# Autodesk Inventor assembly: EnsambleCuerpo
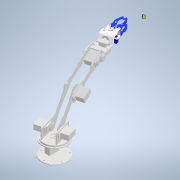
[picture p0: Inventor's stored thumbnail of the model, 180x180]
Saved by Autodesk Inventor 2022 (Build 260153000, 153)
## iProperties
Created: 2021-09-09
Part Number: EnsambleCuerpo
Document SubType Name: Assembly
Designer: Administrador
Author: Administrador
## Documents named in this file (19)
- C:\Users\Administrador\Desktop\Octavo Semestre\Robótica Industrial\Robot\Cuerpo\EnsambleCuerpo.iam
- C:\Users\Administrador\Desktop\Octavo Semestre\Robótica Industrial\Robot\Cuerpo\PartesCuerpo\Base_Suelo.ipt
- C:\Users\Administrador\Desktop\Octavo Semestre\Robótica Industrial\Robot\Cuerpo\PartesCuerpo\Base2.ipt
- C:\Users\Administrador\Desktop\Octavo Semestre\Robótica Industrial\Robot\Cuerpo\PartesCuerpo\Motor Mg995.ipt
- C:\Users\Administrador\Desktop\Octavo Semestre\Robótica Industrial\Robot\Cuerpo\PartesCuerpo\Base3.ipt
- C:\Users\Administrador\Desktop\Octavo Semestre\Robótica Industrial\Robot\Cuerpo\PartesCuerpo\Circulo_Inferior.ipt
- C:\Users\Administrador\Desktop\Octavo Semestre\Robótica Industrial\Robot\Cuerpo\PartesCuerpo\Base4.ipt
- C:\Users\Administrador\Desktop\Octavo Semestre\Robótica Industrial\Robot\Cuerpo\PartesCuerpo\BaseMotoresHombrp.ipt
- C:\Users\Administrador\Desktop\Octavo Semestre\Robótica Industrial\Robot\Cuerpo\PartesCuerpo\Brazo1.1.ipt
- C:\Users\Administrador\Desktop\Octavo Semestre\Robótica Industrial\Robot\Cuerpo\PartesCuerpo\Estella Servo1.ipt
- C:\Users\Administrador\Desktop\Octavo Semestre\Robótica Industrial\Robot\Cuerpo\PartesCuerpo\Brazo2Izquierda.ipt
- C:\Users\Administrador\Desktop\Octavo Semestre\Robótica Industrial\Robot\Cuerpo\PartesCuerpo\Brazo1Izquierda.ipt
- C:\Users\Administrador\Desktop\Octavo Semestre\Robótica Industrial\Robot\Cuerpo\PartesCuerpo\Brazo2Derecha.ipt
- C:\Users\Administrador\Desktop\Octavo Semestre\Robótica Industrial\Robot\Cuerpo\PartesCuerpo\Brazo3Izquierda.ipt
- C:\Users\Administrador\Desktop\Octavo Semestre\Robótica Industrial\Robot\Cuerpo\PartesCuerpo\Brazo3.ipt
- C:\Users\Administrador\Desktop\Octavo Semestre\Robótica Industrial\Robot\Cuerpo\PartesCuerpo\Muñeca1.ipt
- C:\Users\Administrador\Desktop\Octavo Semestre\Robótica Industrial\Robot\Cuerpo\PartesCuerpo\Muñeca2.ipt
- C:\Users\Administrador\Desktop\Octavo Semestre\Robótica Industrial\Robot\Cuerpo\PartesCuerpo\Microservo Mg90.ipt
- C:\Users\Administrador\Desktop\Octavo Semestre\Robótica Industrial\Robot\Pinza\Ensamble Pinza.iam
## Components (26 placed, 18 different names)
1. Base3:1 — Mate:6, Mate:7, Mate:8, Mate:9, Rigid:16, Mate:11, Mate:12
2. Circulo_Inferior:1 — Mate:7, Mate:8, Mate:9, Rigid:16, Rotational:1, Mate:10
3. Base4:1 — Mate:10, Mate:11, Mate:12, Mate:13, Mate:14, Mate:15
4. Base_Suelo:1 — Rigid:15
5. Base2:1 — Rigid:15, Mate:1, Mate:2, Mate:3, Mate:4, Mate:5
6. Motor Mg995:1 — Mate:1, Mate:2, Mate:3, Mate:4, Mate:5, Mate:6, Rotational:1
7. BaseMotoresHombrp:1 — Mate:13, Mate:14, Mate:15, Mate:16, Mate:17, Mate:18, Mate:19, Mate:20, Mate:21
8. Motor Mg995:2 — Mate:16, Mate:17, Mate:18, Mate:22, Rotational:2
9. Motor Mg995:3 — Mate:19, Mate:20, Mate:21, Rotational:4
10. Brazo1.1:1 — Mate:23, Mate:24, Mate:27, Mate:45, Rotational:8
11. Estella Servo1:1 — Mate:22, Mate:23, Mate:24, Rotational:2, Mate:26
12. Brazo2Izquierda:1 — Mate:36, Mate:40, Rotational:6, Mate:45, Rotational:8
13. Brazo1Izquierda:1 — Mate:26, Mate:27, Mate:28, Mate:29, Mate:33, Mate:34, Mate:35
14. Estella Servo1:2 — Mate:28, Mate:29, Rotational:4
15. Brazo2Derecha:1 — Mate:30, Mate:31, Mate:32, Mate:36, Mate:37, Mate:38, Mate:39
16. Motor Mg995:4 — Mate:30, Mate:31, Mate:32, Mate:33, Rotational:5
17. Circulo_Inferior:2 — Mate:34, Mate:35, Rotational:5
18. Motor Mg995:5 — Mate:37, Mate:38, Mate:39, Mate:42, Rotational:7
19. Brazo3Izquierda:1 — Mate:40, Rotational:6, Mate:46
20. Brazo3:1 — Mate:41, Mate:42, Mate:43, Mate:46, Flush:1, Mate:47, Mate:48, Mate:50
21. Circulo_Inferior:4 — Mate:41, Mate:43, Rotational:7
22. Muñeca1:1 — Flush:1, Mate:47, Mate:48, Mate:49, Flush:2
23. Muñeca2:1 — Mate:51, Flush:3
24. Microservo Mg90:1 — Mate:49, Mate:50, Flush:2, Mate:51, Flush:3, Mate:53, Rotational:9
25. Ensamble Pinza:1 [sub-assembly] — Mate:52, Rigid:17
26. Estella Servo1:3 — Mate:52, Mate:53, Rotational:9, Rigid:17
## Relationships (65: Mate 51, RevoluteJoint 8, WeldJoint 3, Flush 3)
- Rigid:15 [WeldJoint] (54 mm): Base_Suelo:1 ↔ Base2:1
- Mate:1: Base2:1 ↔ Motor Mg995:1
- Mate:2: Base2:1 ↔ Motor Mg995:1
- Mate:3: Base2:1 ↔ Motor Mg995:1
- Mate:4: Base2:1 ↔ Motor Mg995:1
- Mate:5: Base2:1 ↔ Motor Mg995:1
- Mate:6: Base3:1 ↔ Motor Mg995:1
- Mate:7: Base3:1 ↔ Circulo_Inferior:1
- Mate:8: Base3:1 ↔ Circulo_Inferior:1
- Mate:9: Base3:1 ↔ Circulo_Inferior:1
- Rigid:16 [WeldJoint]: Base3:1 ↔ Circulo_Inferior:1
- Rotational:1 [RevoluteJoint]: Circulo_Inferior:1 ↔ Motor Mg995:1
- Mate:10: Circulo_Inferior:1 ↔ Base4:1
- Mate:11: Base3:1 ↔ Base4:1
- Mate:12: Base3:1 ↔ Base4:1
- Mate:13: Base4:1 ↔ BaseMotoresHombrp:1
- Mate:14: Base4:1 ↔ BaseMotoresHombrp:1
- Mate:15: Base4:1 ↔ BaseMotoresHombrp:1
- Mate:16: BaseMotoresHombrp:1 ↔ Motor Mg995:2
- Mate:17: BaseMotoresHombrp:1 ↔ Motor Mg995:2
- Mate:18: BaseMotoresHombrp:1 ↔ Motor Mg995:2
- Mate:19: BaseMotoresHombrp:1 ↔ Motor Mg995:3
- Mate:20: BaseMotoresHombrp:1 ↔ Motor Mg995:3
- Mate:21: BaseMotoresHombrp:1 ↔ Motor Mg995:3
- Mate:22: Motor Mg995:2 ↔ Estella Servo1:1
- Mate:23: Brazo1.1:1 ↔ Estella Servo1:1
- Mate:24: Brazo1.1:1 ↔ Estella Servo1:1
- Rotational:2 [RevoluteJoint]: Motor Mg995:2 ↔ Estella Servo1:1
- Mate:26: Estella Servo1:1 ↔ Brazo1Izquierda:1
- Mate:27: Brazo1.1:1 ↔ Brazo1Izquierda:1
- Mate:28: Brazo1Izquierda:1 ↔ Estella Servo1:2
- Mate:29: Brazo1Izquierda:1 ↔ Estella Servo1:2
- Rotational:4 [RevoluteJoint]: Motor Mg995:3 ↔ Estella Servo1:2
- Mate:30: Brazo2Derecha:1 ↔ Motor Mg995:4
- Mate:31: Brazo2Derecha:1 ↔ Motor Mg995:4
- Mate:32: Brazo2Derecha:1 ↔ Motor Mg995:4
- Mate:33: Brazo1Izquierda:1 ↔ Motor Mg995:4
- Mate:34: Brazo1Izquierda:1 ↔ Circulo_Inferior:2
- Mate:35: Brazo1Izquierda:1 ↔ Circulo_Inferior:2
- Rotational:5 [RevoluteJoint]: Motor Mg995:4 ↔ Circulo_Inferior:2
- Mate:36: Brazo2Izquierda:1 ↔ Brazo2Derecha:1
- Mate:37: Brazo2Derecha:1 ↔ Motor Mg995:5
- Mate:38: Brazo2Derecha:1 ↔ Motor Mg995:5
- Mate:39: Brazo2Derecha:1 ↔ Motor Mg995:5
- Mate:40: Brazo2Izquierda:1 ↔ Brazo3Izquierda:1
- Rotational:6 [RevoluteJoint]: Brazo2Izquierda:1 ↔ Brazo3Izquierda:1
- Mate:41: Brazo3:1 ↔ Circulo_Inferior:4
- Mate:42: Motor Mg995:5 ↔ Brazo3:1
- Mate:43: Brazo3:1 ↔ Circulo_Inferior:4
- Rotational:7 [RevoluteJoint]: Motor Mg995:5 ↔ Circulo_Inferior:4
- Mate:45: Brazo1.1:1 ↔ Brazo2Izquierda:1
- Rotational:8 [RevoluteJoint]: Brazo1.1:1 ↔ Brazo2Izquierda:1
- Mate:46: Brazo3Izquierda:1 ↔ Brazo3:1
- Flush:1: Brazo3:1 ↔ Muñeca1:1
- Mate:47: Brazo3:1 ↔ Muñeca1:1
- Mate:48: Brazo3:1 ↔ Muñeca1:1
- Mate:49: Muñeca1:1 ↔ Microservo Mg90:1
- Mate:50 (13 mm): Brazo3:1 ↔ Microservo Mg90:1
- Flush:2: Muñeca1:1 ↔ Microservo Mg90:1
- Mate:51: Muñeca2:1 ↔ Microservo Mg90:1
- Flush:3 (4.3 mm): Muñeca2:1 ↔ Microservo Mg90:1
- Mate:52: Ensamble Pinza:1 ↔ Estella Servo1:3
- Mate:53: Microservo Mg90:1 ↔ Estella Servo1:3
- Rotational:9 [RevoluteJoint]: Microservo Mg90:1 ↔ Estella Servo1:3
- Rigid:17 [WeldJoint]: Ensamble Pinza:1 ↔ Estella Servo1:3
